# Autodesk Inventor assembly: Сборка2
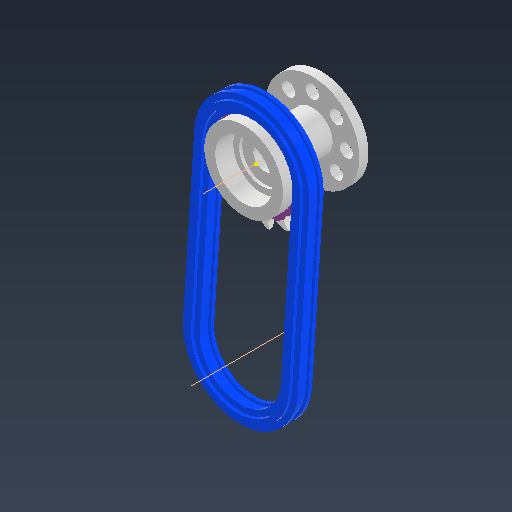
[picture p0: Inventor's stored thumbnail of the model, 512x512]
Saved by Autodesk Inventor 2025 (Build 290162000, 162)
## iProperties
Created: 2024-09-17
Part Number: Сборка2
Document SubType Name: Assembly
Designer: GameHD
Author: GameHD
## Documents named in this file (3)
- C:\Users\GameHD\Desktop\phantom 16950\звезда и втулка.iam
- C:\Users\GameHD\Desktop\phantom 16950\втулка для подш.ipt
- C:\Users\GameHD\Desktop\phantom 16950\цепь короткая 2.0.ipt
## Components (2 placed, 2 different names)
1. втулка для подш:1 — Совмещение:1, Заподлицо:1
2. цепь короткая 2.0:1 — Совмещение:1, Заподлицо:1
## Relationships (2: Mate 1, Flush 1)
- Совмещение:1 [Mate]: втулка для подш:1 ↔ цепь короткая 2.0:1
- Заподлицо:1 [Flush] (4 mm): втулка для подш:1 ↔ цепь короткая 2.0:1
